# Autodesk Inventor assembly: Z
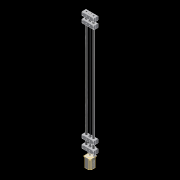
[picture p0: Inventor's stored thumbnail of the model, 180x180]
Saved by Autodesk Inventor 2016 (Build 200138000, 138)
## iProperties
Created: 2017-07-13
Part Number: Z
Document SubType Name: Assembly
Designer: ludwi
Author: ludwi
## Documents named in this file (8)
- H:\MARQ\3D\AXIS_DEV_EDT_V3\X.iam
- H:\MARQ\3D\AXIS_DEV_EDT_V3\AXB.ipt
- C:\Users\ludwi\OneDrive\Documentos\Inventor\Content Center Files\R2016\en-US\DIN BEARING(1)\DIN 625 SKF - SKF 626.ipt
- C:\Users\ludwi\OneDrive\Documentos\Inventor\Content Center Files\R2016\en-US\DIN 935\DIN 935 T1 - M6 x 1 x 10.ipt
- H:\MARQ\3D\AXIS_DEV_EDT_V3\NEMA23.ipt
- H:\MARQ\3D\AXIS_DEV_EDT_V3\MSUP.ipt
- H:\MARQ\3D\AXIS_DEV_EDT_V3\TuboEstructura L.ipt
- H:\MARQ\3D\AXIS_DEV_EDT_V3\M6SL.ipt
## Components (17 placed, 7 different names)
1. AXB:1 — Insert:9, Insert:27, Insert:28
2. AXB:2 — Insert:29
3. AXB:3 — Insert:10, Insert:30
4. AXB:4
5. DIN 625 SKF SKF 626:1 — Insert:9, Mate:6
6. DIN 625 SKF SKF 626:2 — Insert:10, Mate:4
7. DIN 935 M6:1 — Mate:4
8. DIN 935 M6:2 — Mate:6
9. NEMA23:1 — Insert:13, Insert:14, Insert:31
10. MSUP:2 — Insert:13, Insert:14
11. AXB:5 — Mate:14, Flush:3
12. AXB:6 — Mate:7, Mate:8, Flush:3
13. AXB:7 — Mate:12, Flush:1, Flush:2
14. AXB:8 — Mate:11, Mate:13, Flush:1, Flush:2
15. TuboEstructura L:1 — Insert:28, Insert:29, Mate:7, Mate:13, Mate:14
16. TuboEstructura L:2 — Insert:27, Insert:30, Mate:8, Mate:11, Mate:12
17. M6SL:1 — Insert:31
## Relationships (20: Insert 9, Mate 8, Flush 3)
- Insert:9: AXB:1 ↔ DIN 625 SKF SKF 626:1
- Insert:10: AXB:3 ↔ DIN 625 SKF SKF 626:2
- Mate:4: DIN 625 SKF SKF 626:2 ↔ DIN 935 M6:1
- Mate:6: DIN 625 SKF SKF 626:1 ↔ DIN 935 M6:2
- Insert:13: NEMA23:1 ↔ MSUP:2
- Insert:14: NEMA23:1 ↔ MSUP:2
- Insert:27: AXB:1 ↔ TuboEstructura L:2
- Insert:28: AXB:1 ↔ TuboEstructura L:1
- Insert:29: AXB:2 ↔ TuboEstructura L:1
- Insert:30: AXB:3 ↔ TuboEstructura L:2
- Mate:7: AXB:6 ↔ TuboEstructura L:1
- Mate:8: AXB:6 ↔ TuboEstructura L:2
- Mate:11: AXB:8 ↔ TuboEstructura L:2
- Insert:31: NEMA23:1 ↔ M6SL:1
- Mate:12: AXB:7 ↔ TuboEstructura L:2
- Mate:13: AXB:8 ↔ TuboEstructura L:1
- Flush:1: AXB:7 ↔ AXB:8
- Flush:2: AXB:7 ↔ AXB:8
- Mate:14: AXB:5 ↔ TuboEstructura L:1
- Flush:3: AXB:5 ↔ AXB:6
